# Autodesk Inventor assembly: Casev1
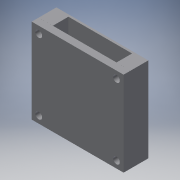
[picture p0: Inventor's stored thumbnail of the model, 180x180]
Saved by Autodesk Inventor 2017 (Build 210142000, 142)
## iProperties
Created: 2020-01-28
Part Number: Casev1
Document SubType Name: Assembly
Designer: Manny
Author: Manny
## Documents named in this file (3)
- C:\Users\Owner\Documents\ENG Year 5\Casev1.iam
- C:\Users\Owner\Documents\ENG Year 5\Case_Top_Partv1.ipt
- C:\Users\Owner\Documents\ENG Year 5\Bottom_part.ipt
## Components (2 placed, 2 different names)
1. Case_Top_Partv1:1 — Flush:1, Flush:2, Mate:1
2. Bottom_part:1 — Flush:1, Flush:2, Mate:1
## Relationships (3: Flush 2, Mate 1)
- Flush:1: Case_Top_Partv1:1 ↔ Bottom_part:1
- Flush:2: Case_Top_Partv1:1 ↔ Bottom_part:1
- Mate:1: Case_Top_Partv1:1 ↔ Bottom_part:1
